# Autodesk Inventor assembly: Base2
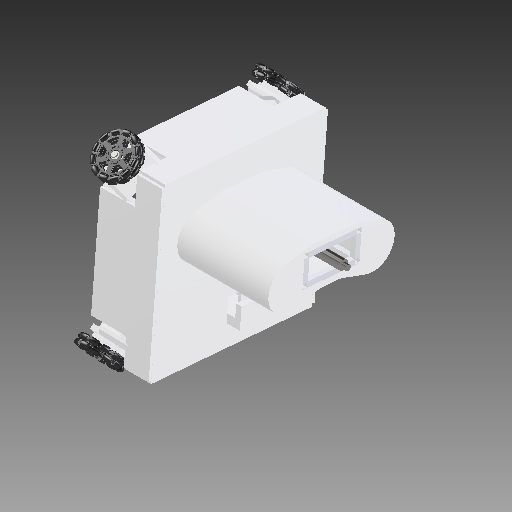
[picture p0: Inventor's stored thumbnail of the model, 512x512]
Saved by Autodesk Inventor 2017 SP1 (Build 210196100, 196)
## iProperties
Created: 2017-06-13
Part Number: Base2
Document SubType Name: Assembly
Designer: zallen
Author: zallen
## Documents named in this file (7)
- C:\Users\Zach\Documents\GitHub\cr-laundry-robot\src\Base\Base.iam
- C:\Users\Zach\Documents\GitHub\cr-laundry-robot\src\Base\Chassis\Chassis.iam
- C:\Users\Zach\Documents\GitHub\cr-laundry-robot\lib\Linear Actuator 450mm\LinearActuator450mm.iam
- C:\Users\Zach\Documents\GitHub\cr-laundry-robot\src\Base\Riser Base.ipt
- C:\Users\Zach\Documents\GitHub\cr-laundry-robot\src\Base\Top Cover.ipt
- C:\Users\Zach\Documents\GitHub\cr-laundry-robot\src\Base\Front Cover.ipt
- C:\Users\Zach\Documents\GitHub\cr-laundry-robot\src\Base\Wheel Assembly\Wheel Assembly.iam
## Components (12 placed, 6 different names)
1. Chassis:1 [sub-assembly] — Mate:17, Mate:18, Mate:19, Mate:20, Mate:23, Mate:25, Mate:28, Mate:29, Mate:30, Mate:33, Mate:36, Mate:37, Mate:38, Mate:39, Mate:40, Mate:41, Mate:42, Mate:43, Mate:44, Mate:45, Mate:46, Mate:47, Mate:48, Mate:49
2. LinearActuator450mm:1 [sub-assembly] — Mate:17
3. Riser Base:1 — Mate:18, Mate:19, Mate:20, Mate:21, Mate:22
4. Top Cover:1 — Mate:21, Mate:22, Mate:23, Mate:24, Mate:26, Mate:27, Mate:31, Mate:32, Mate:34
5. Front Cover:1 — Mate:24, Mate:25, Mate:26, Mate:35
6. Front Cover:2 — Mate:27, Mate:28, Mate:29
7. Front Cover:3 — Mate:33, Mate:34, Mate:35
8. Front Cover:4 — Mate:30, Mate:31, Mate:32
9. Wheel Assembly:1 [sub-assembly] — Mate:36, Mate:37, Mate:38, Mate:39, Mate:40
10. Wheel Assembly:2 [sub-assembly] — Mate:41, Mate:42, Mate:43
11. Wheel Assembly:3 [sub-assembly] — Mate:44, Mate:45, Mate:46
12. Wheel Assembly:4 [sub-assembly] — Mate:47, Mate:48, Mate:49
## Relationships (33: Mate 33)
- Mate:17: Chassis:1 ↔ LinearActuator450mm:1
- Mate:18: Chassis:1 ↔ Riser Base:1
- Mate:19: Chassis:1 ↔ Riser Base:1
- Mate:20: Chassis:1 ↔ Riser Base:1
- Mate:21: Riser Base:1 ↔ Top Cover:1
- Mate:22: Riser Base:1 ↔ Top Cover:1
- Mate:23: Chassis:1 ↔ Top Cover:1
- Mate:24: Top Cover:1 ↔ Front Cover:1
- Mate:25: Chassis:1 ↔ Front Cover:1
- Mate:26: Top Cover:1 ↔ Front Cover:1
- Mate:27: Top Cover:1 ↔ Front Cover:2
- Mate:28: Chassis:1 ↔ Front Cover:2
- Mate:29: Chassis:1 ↔ Front Cover:2
- Mate:30: Chassis:1 ↔ Front Cover:4
- Mate:31: Top Cover:1 ↔ Front Cover:4
- Mate:32: Top Cover:1 ↔ Front Cover:4
- Mate:33: Chassis:1 ↔ Front Cover:3
- Mate:34: Top Cover:1 ↔ Front Cover:3
- Mate:35: Front Cover:1 ↔ Front Cover:3
- Mate:36: Chassis:1 ↔ Wheel Assembly:1
- Mate:37: Chassis:1 ↔ Wheel Assembly:1
- Mate:38: Chassis:1 ↔ Wheel Assembly:1
- Mate:39: Chassis:1 ↔ Wheel Assembly:1
- Mate:40: Chassis:1 ↔ Wheel Assembly:1
- Mate:41: Chassis:1 ↔ Wheel Assembly:2
- Mate:42: Chassis:1 ↔ Wheel Assembly:2
- Mate:43: Chassis:1 ↔ Wheel Assembly:2
- Mate:44: Chassis:1 ↔ Wheel Assembly:3
- Mate:45: Chassis:1 ↔ Wheel Assembly:3
- Mate:46: Chassis:1 ↔ Wheel Assembly:3
- Mate:47: Chassis:1 ↔ Wheel Assembly:4
- Mate:48: Chassis:1 ↔ Wheel Assembly:4
- Mate:49: Chassis:1 ↔ Wheel Assembly:4
